# Autodesk Inventor assembly: sea_trash_collector
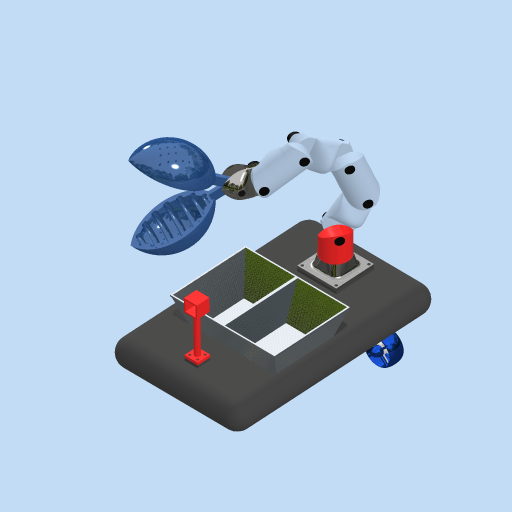
[picture p0: Inventor's stored thumbnail of the model, 512x512]
Saved by Autodesk Inventor 2023 (Build 270158000, 158)
## iProperties
Created: 2024-11-14
Part Number: sea_trash_collector
Document SubType Name: Assembly
Designer: ADMIN
Author: ADMIN
## Documents named in this file (12)
- C:\Users\ADMIN\Documents\MECHATRONICS\sea_trash\sea_trash_collector.iam
- C:\Users\ADMIN\Documents\MECHATRONICS\sea_trash\hull.ipt
- C:\Users\ADMIN\Documents\MECHATRONICS\sea_trash\base_link0.ipt
- C:\Users\ADMIN\Documents\MECHATRONICS\sea_trash\link1.ipt
- C:\Users\ADMIN\Documents\MECHATRONICS\sea_trash\link2.ipt
- C:\Users\ADMIN\Documents\MECHATRONICS\sea_trash\head_link.ipt
- C:\Users\ADMIN\Documents\MECHATRONICS\sea_trash\gripper.ipt
- C:\Users\ADMIN\Documents\MECHATRONICS\sea_trash\joint.ipt
- C:\Users\ADMIN\Documents\MECHATRONICS\sea_trash\small_gripper.ipt
- C:\Users\ADMIN\Documents\MECHATRONICS\sea_trash\tray.ipt
- C:\Users\ADMIN\Documents\MECHATRONICS\sea_trash\camera_pole.ipt
- C:\Users\ADMIN\Documents\MECHATRONICS\sea_trash\ThrusterAssembly.iam
## Components (20 placed, 11 different names)
1. hull:1 — Mate:1, Mate:2, Mate:3, Mate:26, Mate:27, Mate:28, Mate:29, Mate:30, Mate:31, Flush:7, Flush:8, Flush:9, Flush:10, Flush:11, Flush:12
2. base_link0:1 — Mate:1, Mate:2, Mate:3, Mate:4, Mate:5
3. link1:1 — Mate:4, Mate:5, Mate:6, Mate:7
4. link2:1 — Mate:6, Mate:7, Mate:8, Mate:9, Mate:20, Flush:1, Mate:21, Flush:2
5. link2:2 — Mate:10, Mate:11, Mate:12, Mate:13, Mate:22, Mate:23, Flush:3, Flush:4
6. link2:3 — Mate:12, Mate:13, Mate:14, Mate:15
7. link2:4 — Mate:8, Mate:9, Mate:10, Mate:11
8. head_link:1 — Mate:14, Mate:15, Mate:16, Mate:17, Mate:18, Mate:19, Mate:24, Mate:25, Flush:5, Flush:6
9. gripper:1 — Mate:16, Mate:17
10. gripper:2 — Mate:18, Mate:19
11. joint:1 — Mate:20, Flush:1
12. joint:2 — Mate:21, Flush:2
13. joint:3 — Mate:22, Flush:3
14. joint:4 — Mate:23, Flush:4
15. joint:5 — Mate:24, Flush:5
16. small_gripper:1 — Mate:25, Flush:6
17. tray:1 — Mate:26, Mate:27, Mate:28
18. camera_pole:1 — Mate:29, Mate:30, Mate:31
19. ThrusterAssembly:2 [sub-assembly] — Flush:7, Flush:8, Flush:9
20. ThrusterAssembly:3 [sub-assembly] — Flush:10, Flush:11, Flush:12
## Relationships (43: Mate 31, Flush 12)
- Mate:1: hull:1 ↔ base_link0:1
- Mate:2: hull:1 ↔ base_link0:1
- Mate:3: hull:1 ↔ base_link0:1
- Mate:4: base_link0:1 ↔ link1:1
- Mate:5: base_link0:1 ↔ link1:1
- Mate:6: link1:1 ↔ link2:1
- Mate:7: link1:1 ↔ link2:1
- Mate:8: link2:1 ↔ link2:4
- Mate:9: link2:1 ↔ link2:4
- Mate:10: link2:2 ↔ link2:4
- Mate:11: link2:2 ↔ link2:4
- Mate:12: link2:2 ↔ link2:3
- Mate:13: link2:2 ↔ link2:3
- Mate:14: link2:3 ↔ head_link:1
- Mate:15: link2:3 ↔ head_link:1
- Mate:16: head_link:1 ↔ gripper:1
- Mate:17: head_link:1 ↔ gripper:1
- Mate:18: head_link:1 ↔ gripper:2
- Mate:19: head_link:1 ↔ gripper:2
- Mate:20: link2:1 ↔ joint:1
- Flush:1 (50 mm): link2:1 ↔ joint:1
- Mate:21: link2:1 ↔ joint:2
- Mate:22: link2:2 ↔ joint:3
- Mate:23: link2:2 ↔ joint:4
- Mate:24: head_link:1 ↔ joint:5
- Mate:25: head_link:1 ↔ small_gripper:1
- Flush:2 (50 mm): link2:1 ↔ joint:2
- Flush:3 (50 mm): link2:2 ↔ joint:3
- Flush:4 (50 mm): link2:2 ↔ joint:4
- Flush:5 (50 mm): head_link:1 ↔ joint:5
- Flush:6 (33 mm): head_link:1 ↔ small_gripper:1
- Mate:26: hull:1 ↔ tray:1
- Mate:27: hull:1 ↔ tray:1
- Mate:28: hull:1 ↔ tray:1
- Mate:29: hull:1 ↔ camera_pole:1
- Mate:30: hull:1 ↔ camera_pole:1
- Mate:31: hull:1 ↔ camera_pole:1
- Flush:7: hull:1 ↔ ThrusterAssembly:2
- Flush:8: hull:1 ↔ ThrusterAssembly:2
- Flush:9 (17 mm): hull:1 ↔ ThrusterAssembly:2
- Flush:10: hull:1 ↔ ThrusterAssembly:3
- Flush:11: hull:1 ↔ ThrusterAssembly:3
- Flush:12 (-17 mm): hull:1 ↔ ThrusterAssembly:3
